# Autodesk Inventor assembly: assy.0032
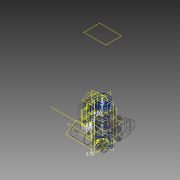
[picture p0: Inventor's stored thumbnail of the model, 180x180]
Saved by Autodesk Inventor 2015 (Build 190159000, 159)
## iProperties
Created: 2015-08-29
Document SubType Name: Assembly
Designer: Frank Conroy
Mass: 406.806 g
Surface Area: 819.776 cm^2
Volume: 203.089 cm^3
Density: 2.0031 g/cm^3
Description: GA
Author: Frank Conroy
## Documents named in this file (20)
- C:\Users\francis\Documents\GitHub\CAD\assy.iam
- C:\Users\francis\Documents\GitHub\CAD\throttle_ETC.ipt
- C:\Users\francis\Documents\GitHub\CAD\bearing.ipt
- C:\Users\francis\Documents\GitHub\CAD\crouzet_motor.ipt
- C:\Users\francis\Documents\GitHub\CAD\Bosch TPS 2\Workspaces\Workspace\Bosch TPS.ipt
- C:\Users\francis\Documents\GitHub\CAD\pulley_5mm.ipt
- C:\Users\francis\Documents\GitHub\CAD\pulley_8mm.ipt
- C:\Users\francis\Documents\GitHub\CAD\motor_plate.ipt
- C:\Users\francis\Documents\GitHub\CAD\pulley_plate.ipt
- C:\Users\francis\Documents\GitHub\CAD\spring_arm.ipt
- C:\Users\francis\Documents\Inventor\Content Center Files\R2015\en-US\ANSI B18.3.4M(1)\ANSI B18.3.4M - M4 x 0.7 x 6(2).ipt
- C:\Users\francis\Documents\GitHub\CAD\butterfly.ipt
- C:\Users\francis\Documents\GitHub\CAD\ghost.ipt
- C:\Users\francis\Documents\GitHub\CAD\STANDOFF2.ipt
- C:\Users\francis\Documents\GitHub\CAD\STANDOFF3.ipt
- C:\Users\francis\Documents\GitHub\CAD\OPENSTOPBRKT.ipt
- C:\Users\francis\Documents\GitHub\CAD\CLOSESTOPBRKT.ipt
- C:\Users\francis\Documents\Inventor\Content Center Files\R2015\en-US\ANSI B18.3.4M(2)\ANSI B18.3.4M - M4 x 0.7 x 35(1).ipt
- C:\Users\francis\Documents\Inventor\Content Center Files\R2015\en-US\ANSI B18.3.4M(2)\ANSI B18.3.4M - M3 x 0.5 x 8(1).ipt
- C:\Users\francis\Documents\Inventor\Content Center Files\R2015\en-US\ANSI B18.3.4M(2)\ANSI B18.3.4M - M3 x 0.5 x 25(1).ipt
## Components (31 placed, 19 different names)
1. throttle_ETC:1 — Mate:1, Mate:2, Mate:3, Mate:4, Mate:5, Angle:1, Angle:3, Symmetry:1, Angle:5, Flush:1, Mate:20, Mate:21, Mate:22, Flush:2, Mate:23, Flush:4, Mate:25, Mate:27, Flush:28, Flush:29, Mate:40
2. bearing:1 — Mate:2, Mate:3, Mate:6
3. bearing:2 — Mate:4, Mate:5, Mate:7, Mate:9
4. crouzet_motor:1 — Flush:1, Mate:19, Mate:21, Mate:22, Angle:6
5. Bosch TPS:1 — Angle:1, Mate:6, Mate:23, Insert:5, Insert:6
6. Bosch TPS:2 — Angle:3, Mate:7, Mate:24, Insert:1, Insert:2
7. pulley_5mm:1 — Mate:19, Flush:3
8. pulley_8mm:1 — Mate:20, Flush:3
9. motor_plate:1 — Flush:2, Mate:24, Flush:38, Flush:39, Flush:40, Flush:41, Mate:41, Mate:42, Mate:43, Mate:44, Mate:45, Mate:46, Mate:47, Mate:48
10. pulley_plate:1 — Flush:4, Flush:42, Flush:43, Flush:45, Flush:46
11. spring_arm:1 — Mate:25, Flush:27, Mate:27, Mate:36, Mate:37, Mate:38, Mate:39, Flush:33, Flush:34
12. Broached Hexagon Socket Button Head Cap Screw - Metric M4 x 0.7 x 6:1 — Mate:36, Mate:37
13. Broached Hexagon Socket Button Head Cap Screw - Metric M4 x 0.7 x 6:2 — Mate:38, Mate:39
14. butterfly:1 — Flush:28, Flush:29, Flush:30, Mate:40
15. ghost:1 — Flush:33, Flush:34, Flush:44
16. STANDOFF2:1 — Flush:38, Flush:39
17. STANDOFF3:1 — Flush:40, Flush:41
18. OPENSTOPBRKT:1 — Flush:42, Flush:43, Flush:44, Flush:47, Mate:49, Mate:50, Mate:51, Mate:52
19. CLOSESTOPBRKT:1 — Flush:45, Flush:46, Flush:47, Insert:3, Insert:4
20. Forged Hexagon Socket Button Head Cap Screw - Metric M4 x 0.7 x 35:1 — Insert:1
21. Forged Hexagon Socket Button Head Cap Screw - Metric M4 x 0.7 x 35:2 — Insert:2
22. Forged Hexagon Socket Button Head Cap Screw - Metric M3 x 0.5 x 8:1 — Mate:41, Mate:42
23. Forged Hexagon Socket Button Head Cap Screw - Metric M3 x 0.5 x 8:2 — Mate:43, Mate:44
24. Forged Hexagon Socket Button Head Cap Screw - Metric M3 x 0.5 x 8:3 — Mate:45, Mate:46
25. Forged Hexagon Socket Button Head Cap Screw - Metric M3 x 0.5 x 8:4 — Mate:47, Mate:48
26. Forged Hexagon Socket Button Head Cap Screw - Metric M3 x 0.5 x 25:1 — Insert:3
27. Forged Hexagon Socket Button Head Cap Screw - Metric M3 x 0.5 x 25:2 — Insert:4
28. Forged Hexagon Socket Button Head Cap Screw - Metric M3 x 0.5 x 25:3 — Mate:49, Mate:50
29. Forged Hexagon Socket Button Head Cap Screw - Metric M3 x 0.5 x 25:4 — Mate:51, Mate:52
30. Forged Hexagon Socket Button Head Cap Screw - Metric M4 x 0.7 x 35:3 — Insert:5
31. Forged Hexagon Socket Button Head Cap Screw - Metric M4 x 0.7 x 35:4 — Insert:6
## Relationships (66: Mate 35, Flush 20, Insert 6, Angle 4, Symmetry 1)
- Mate:1: throttle_ETC:1
- Mate:2: throttle_ETC:1 ↔ bearing:1
- Mate:3: throttle_ETC:1 ↔ bearing:1
- Mate:4: throttle_ETC:1 ↔ bearing:2
- Mate:5: throttle_ETC:1 ↔ bearing:2
- Angle:1 (0 deg): throttle_ETC:1 ↔ Bosch TPS:1
- Angle:3 (180 deg): throttle_ETC:1 ↔ Bosch TPS:2
- Mate:6: bearing:1 ↔ Bosch TPS:1
- Mate:7: bearing:2 ↔ Bosch TPS:2
- Symmetry:1: throttle_ETC:1
- Mate:9: bearing:2
- Mate:10
- Angle:5 (90 deg): throttle_ETC:1
- Mate:13 (48.6 mm)
- Flush:1: throttle_ETC:1 ↔ crouzet_motor:1
- Mate:19: crouzet_motor:1 ↔ pulley_5mm:1
- Mate:20: throttle_ETC:1 ↔ pulley_8mm:1
- Mate:21 (49 mm): throttle_ETC:1 ↔ crouzet_motor:1
- Mate:22: throttle_ETC:1 ↔ crouzet_motor:1
- Angle:6 (215 deg): crouzet_motor:1
- Flush:2: throttle_ETC:1 ↔ motor_plate:1
- Flush:3: pulley_5mm:1 ↔ pulley_8mm:1
- Mate:23 (22 mm): throttle_ETC:1 ↔ Bosch TPS:1
- Mate:24 (25 mm): Bosch TPS:2 ↔ motor_plate:1
- Flush:4: throttle_ETC:1 ↔ pulley_plate:1
- Mate:25: throttle_ETC:1 ↔ spring_arm:1
- Flush:27: spring_arm:1
- Mate:27 (12 mm): throttle_ETC:1 ↔ spring_arm:1
- Mate:36: spring_arm:1 ↔ Broached Hexagon Socket Button Head Cap Screw - Metric M4 x 0.7 x 6:1
- Mate:37 (5 mm): spring_arm:1 ↔ Broached Hexagon Socket Button Head Cap Screw - Metric M4 x 0.7 x 6:1
- Mate:38: spring_arm:1 ↔ Broached Hexagon Socket Button Head Cap Screw - Metric M4 x 0.7 x 6:2
- Mate:39 (5 mm): spring_arm:1 ↔ Broached Hexagon Socket Button Head Cap Screw - Metric M4 x 0.7 x 6:2
- Flush:28: throttle_ETC:1 ↔ butterfly:1
- Flush:29: throttle_ETC:1 ↔ butterfly:1
- Flush:30: butterfly:1
- Flush:33: spring_arm:1 ↔ ghost:1
- Flush:34: spring_arm:1 ↔ ghost:1
- Mate:40: throttle_ETC:1 ↔ butterfly:1
- Flush:38: motor_plate:1 ↔ STANDOFF2:1
- Flush:39: motor_plate:1 ↔ STANDOFF2:1
- Flush:40: motor_plate:1 ↔ STANDOFF3:1
- Flush:41: motor_plate:1 ↔ STANDOFF3:1
- Flush:42: pulley_plate:1 ↔ OPENSTOPBRKT:1
- Flush:43: pulley_plate:1 ↔ OPENSTOPBRKT:1
- Flush:44 (-3 mm): ghost:1 ↔ OPENSTOPBRKT:1
- Flush:45: pulley_plate:1 ↔ CLOSESTOPBRKT:1
- Flush:46: pulley_plate:1 ↔ CLOSESTOPBRKT:1
- Flush:47: OPENSTOPBRKT:1 ↔ CLOSESTOPBRKT:1
- Insert:1: Bosch TPS:2 ↔ Forged Hexagon Socket Button Head Cap Screw - Metric M4 x 0.7 x 35:1
- Insert:2: Bosch TPS:2 ↔ Forged Hexagon Socket Button Head Cap Screw - Metric M4 x 0.7 x 35:2
- Mate:41: motor_plate:1 ↔ Forged Hexagon Socket Button Head Cap Screw - Metric M3 x 0.5 x 8:1
- Mate:42: motor_plate:1 ↔ Forged Hexagon Socket Button Head Cap Screw - Metric M3 x 0.5 x 8:1
- Mate:43: motor_plate:1 ↔ Forged Hexagon Socket Button Head Cap Screw - Metric M3 x 0.5 x 8:2
- Mate:44: motor_plate:1 ↔ Forged Hexagon Socket Button Head Cap Screw - Metric M3 x 0.5 x 8:2
- Mate:45: motor_plate:1 ↔ Forged Hexagon Socket Button Head Cap Screw - Metric M3 x 0.5 x 8:3
- Mate:46: motor_plate:1 ↔ Forged Hexagon Socket Button Head Cap Screw - Metric M3 x 0.5 x 8:3
- Mate:47: motor_plate:1 ↔ Forged Hexagon Socket Button Head Cap Screw - Metric M3 x 0.5 x 8:4
- Mate:48: motor_plate:1 ↔ Forged Hexagon Socket Button Head Cap Screw - Metric M3 x 0.5 x 8:4
- Insert:3: CLOSESTOPBRKT:1 ↔ Forged Hexagon Socket Button Head Cap Screw - Metric M3 x 0.5 x 25:1
- Insert:4: CLOSESTOPBRKT:1 ↔ Forged Hexagon Socket Button Head Cap Screw - Metric M3 x 0.5 x 25:2
- Mate:49: OPENSTOPBRKT:1 ↔ Forged Hexagon Socket Button Head Cap Screw - Metric M3 x 0.5 x 25:3
- Mate:50: OPENSTOPBRKT:1 ↔ Forged Hexagon Socket Button Head Cap Screw - Metric M3 x 0.5 x 25:3
- Mate:51: OPENSTOPBRKT:1 ↔ Forged Hexagon Socket Button Head Cap Screw - Metric M3 x 0.5 x 25:4
- Mate:52: OPENSTOPBRKT:1 ↔ Forged Hexagon Socket Button Head Cap Screw - Metric M3 x 0.5 x 25:4
- Insert:5: Bosch TPS:1 ↔ Forged Hexagon Socket Button Head Cap Screw - Metric M4 x 0.7 x 35:3
- Insert:6: Bosch TPS:1 ↔ Forged Hexagon Socket Button Head Cap Screw - Metric M4 x 0.7 x 35:4
